# Autodesk Inventor assembly: Tower Pro 9g Micro Servo SG90_MIR
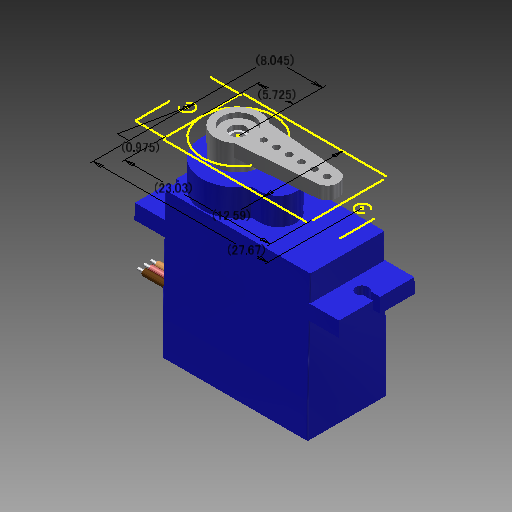
[picture p0: Inventor's stored thumbnail of the model, 512x512]
Saved by Autodesk Inventor 2017 (Build 210142000, 142)
## iProperties
Created: 2015-05-27
Part Number: Tower Pro 9g Micro Servo SG90_MIR
Material: 一般
Document SubType Name: Assembly
Designer: sktom
Author: sktom
Sending System: SolidWorks 2014
Last Author: Simon
Last Saved: 2015-06-03
## Documents named in this file (3)
- D:\OneDrive\CAD\MAJ\hackberry\HACKberry-hardware\3D_69%inlength\Inventor_right\HbHandForChild\servo\Tower Pro 9g Micro Servo SG90_MIR.iam
- D:\OneDrive\CAD\MAJ\hackberry\HACKberry-hardware\3D_69%inlength\Inventor_right\HbHandForChild\servo\Tower Pro 9g Micro Servo SG90_MIR.ipt
- D:\OneDrive\CAD\MAJ\hackberry\HACKberry-hardware\3D_69%inlength\Inventor_right\HbHandForChild\servo\SG90 plastic Horn_MIR.ipt
## Components (2 placed, 2 different names)
1. Tower Pro 9g Micro Servo SG90_MIR:1 — 挿入:1
2. SG90 plastic Horn_MIR:1 — 挿入:1
## Relationships (1: Insert 1)
- 挿入:1 [Insert]: Tower Pro 9g Micro Servo SG90_MIR:1 ↔ SG90 plastic Horn_MIR:1
